# Autodesk Inventor assembly: TR1 Actuator
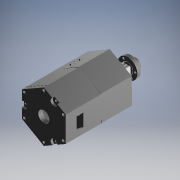
[picture p0: Inventor's stored thumbnail of the model, 180x180]
Saved by Autodesk Inventor 2017 (Build 210142000, 142)
## iProperties
Created: 2018-10-09
Part Number: TR1 Actuator
Document SubType Name: Assembly
Designer: Zach
Mass: 1249.01 g
Surface Area: 2931.11 cm^2
Volume: 1069.5 cm^3
Density: 1.16785 g/cm^3
Author: Zach
## Documents named in this file (21)
- C:\Users\Dell\Documents\GitHub\tr2\Actuator 1.3\Actuator 1.3.iam
- C:\Users\Dell\Documents\GitHub\tr2\Actuator 1.3\TA01.ipt
- C:\Users\Dell\Documents\GitHub\tr2\Actuator 1.3\Arm Actuator\Design Accelerator\Spur Gears2.iam
- C:\Users\Dell\Documents\GitHub\tr2\Actuator 1.3\EMS22XXX-D28-LSX.ipt
- C:\Users\Dell\Documents\GitHub\tr2\Actuator 1.3\12RPM Gear Motor.ipt
- C:\Users\Dell\Documents\GitHub\tr2\Actuator 1.3\Slip Ring.ipt
- C:\Users\Dell\Documents\GitHub\tr2\Actuator 1.3\TA06.ipt
- C:\Users\Dell\Documents\GitHub\tr2\Actuator 1.3\Steel Tubing.ipt
- C:\Users\Dell\Documents\GitHub\tr2\Actuator 1.3\Flange Bearing.ipt
- C:\Users\Dell\Documents\GitHub\tr2\Actuator 1.3\Shaft Collar.ipt
- C:\Users\Dell\Documents\GitHub\tr2\Actuator 1.3\Arm Actuator\Design Accelerator\Spur Gear13.ipt
- C:\Users\Dell\Documents\GitHub\tr2\Actuator 1.3\6mm Mounting Hub, thick.ipt
- C:\Users\Dell\Documents\GitHub\tr2\Actuator 1.3\TA02c.ipt
- C:\Users\Dell\Documents\GitHub\tr2\Actuator 1.3\TA02b.ipt
- C:\Users\Dell\Documents\GitHub\tr2\Actuator 1.3\Bushing.ipt
- C:\Users\Dell\Documents\GitHub\tr2\Actuator 1.3\545340 assembly.iam
- C:\Users\Dell\Documents\GitHub\tr2\Actuator 1.3\TA07.ipt
- C:\Users\Dell\Documents\GitHub\tr2\Actuator 1.3\TA08.ipt
- C:\Users\Dell\Documents\GitHub\tr2\Actuator 1.3\Rubber Square 1 in.ipt
- C:\Users\Dell\Documents\GitHub\tr2\Actuator 1.3\TA11.ipt
- C:\Users\Dell\Documents\Inventor\Content Center Files\R2017\en-US\ISO 4762(2)\ISO 4762 - M4 x 8ISO.ipt
## Components (26 placed, 20 different names)
1. TA01:1 — Mate:130, Mate:161, Mate:184, Mate:197, Mate:198, Mate:199
2. TA06:1 — Mate:34, Mate:35, Mate:82, Mate:83, Mate:129
3. Spur Gears:1 [sub-assembly] — Mate:33, Mate:97, Mate:121, Mate:123, Mate:124, Mate:125, Mate:129
4. 12RPM Gear Motor:1 — Mate:86, Mate:88, Mate:102, Mate:103, Mate:114, Mate:115
5. EMS22XXX-D28-LSX:1 — Mate:118, Mate:126, Angle:1, Mate:134, Mate:203
6. Slip Ring:1 — Mate:33, Mate:34, Mate:35, Mate:83
7. Steel Tubing:1 — Mate:76, Mate:77, Flush:2, Mate:82, Mate:84, Mate:96, Mate:98, Mate:104, Mate:120, Mate:121, Mate:162
8. Flange Bearing:1 — Mate:76, Mate:179
9. Shaft Collar:1 — Mate:77, Flush:2, Mate:180
10. Flange Bearing:2 — Mate:84, Mate:180
11. Spur Gear1:1 — Mate:88, Mate:116
12. 6mm Mounting Hub, thick:1 — Mate:86, Mate:114, Mate:116, Flush:3
13. TA02c:1 — Mate:98, Mate:99, Mate:105, Mate:127, Mate:128, Mate:130, Mate:131, Angle:2, Mate:197, Mate:198, Mate:199
14. TA02b:1 — Mate:96, Mate:97, Mate:99, Mate:102, Mate:103, Mate:115, Mate:126, Angle:1, Mate:131, Mate:132, Mate:133, Mate:134, Mate:179, Mate:185, Mate:187, Mate:188, Mate:189, Mate:190, Mate:191, Mate:193, Mate:194, Mate:195, Mate:196
15. Bushing:1 — Mate:104, Mate:105
16. Spur Gear1:2 — Mate:119
17. 6mm Mounting Hub, thick:2 — Mate:118, Mate:119, Flush:3, Mate:202
18. 545340 assembly:1 [sub-assembly] — Mate:120, Mate:123, Mate:124, Mate:125
19. EMS22XXX-D28-LSX:2 — Mate:127, Mate:128, Angle:2, Mate:135
20. TA07:1 — Mate:132, Mate:133, Mate:136, Mate:183
21. TA08:1 — Mate:135, Mate:136, Mate:183
22. Rubber Square 1 in:1 — Mate:192, Mate:193, Mate:194
23. Rubber Square 1 in:2 — Mate:186, Mate:195, Mate:196
24. TA11:1 — Mate:185, Mate:186, Mate:187, Mate:188
25. TA11:2 — Mate:189, Mate:190, Mate:191, Mate:192
26. ISO 4762 M4 x 8:2 — Mate:202, Mate:203
## Relationships (67: Mate 63, Flush 2, Angle 2)
- Mate:33: Spur Gears:1 ↔ Slip Ring:1
- Mate:34: TA06:1 ↔ Slip Ring:1
- Mate:35: TA06:1 ↔ Slip Ring:1
- Mate:76: Steel Tubing:1 ↔ Flange Bearing:1
- Mate:77: Steel Tubing:1 ↔ Shaft Collar:1
- Flush:2: Steel Tubing:1 ↔ Shaft Collar:1
- Mate:82: TA06:1 ↔ Steel Tubing:1
- Mate:83: TA06:1 ↔ Slip Ring:1
- Mate:84: Steel Tubing:1 ↔ Flange Bearing:2
- Mate:86: 12RPM Gear Motor:1 ↔ 6mm Mounting Hub, thick:1
- Mate:88: 12RPM Gear Motor:1 ↔ Spur Gear1:1
- Mate:96: Steel Tubing:1 ↔ TA02b:1
- Mate:97: Spur Gears:1 ↔ TA02b:1
- Mate:98: Steel Tubing:1 ↔ TA02c:1
- Mate:99: TA02c:1 ↔ TA02b:1
- Mate:102: 12RPM Gear Motor:1 ↔ TA02b:1
- Mate:103: 12RPM Gear Motor:1 ↔ TA02b:1
- Mate:104: Steel Tubing:1 ↔ Bushing:1
- Mate:105: TA02c:1 ↔ Bushing:1
- Mate:114: 12RPM Gear Motor:1 ↔ 6mm Mounting Hub, thick:1
- Mate:115: 12RPM Gear Motor:1 ↔ TA02b:1
- Mate:116: Spur Gear1:1 ↔ 6mm Mounting Hub, thick:1
- [Mate]: Spur Gear1:2 ↔ 6mm Mounting Hub, thick:2
- Mate:118: EMS22XXX-D28-LSX:1 ↔ 6mm Mounting Hub, thick:2
- Mate:119: Spur Gear1:2 ↔ 6mm Mounting Hub, thick:2
- Flush:3: 6mm Mounting Hub, thick:1 ↔ 6mm Mounting Hub, thick:2
- Mate:120: Steel Tubing:1 ↔ 545340 assembly:1
- Mate:121: Spur Gears:1 ↔ Steel Tubing:1
- Mate:123: Spur Gears:1 ↔ 545340 assembly:1
- Mate:124: Spur Gears:1 ↔ 545340 assembly:1
- Mate:125: Spur Gears:1 ↔ 545340 assembly:1
- Mate:126: EMS22XXX-D28-LSX:1 ↔ TA02b:1
- Angle:1 (0 deg): EMS22XXX-D28-LSX:1 ↔ TA02b:1
- Mate:127: TA02c:1 ↔ EMS22XXX-D28-LSX:2
- Mate:128: TA02c:1 ↔ EMS22XXX-D28-LSX:2
- Mate:129: TA06:1 ↔ Spur Gears:1
- Mate:130: TA01:1 ↔ TA02c:1
- Mate:131: TA02c:1 ↔ TA02b:1
- Angle:2 (0 deg): TA02c:1 ↔ EMS22XXX-D28-LSX:2
- Mate:132: TA02b:1 ↔ TA07:1
- Mate:133: TA02b:1 ↔ TA07:1
- Mate:134: EMS22XXX-D28-LSX:1 ↔ TA02b:1
- Mate:135: EMS22XXX-D28-LSX:2 ↔ TA08:1
- Mate:136: TA07:1 ↔ TA08:1
- Mate:161: TA01:1
- Mate:162: Steel Tubing:1
- Mate:179: Flange Bearing:1 ↔ TA02b:1
- Mate:180: Shaft Collar:1 ↔ Flange Bearing:2
- Mate:183: TA07:1 ↔ TA08:1
- Mate:184: TA01:1
- Mate:185: TA02b:1 ↔ TA11:1
- Mate:186: Rubber Square 1 in:2 ↔ TA11:1
- Mate:187: TA02b:1 ↔ TA11:1
- Mate:188: TA02b:1 ↔ TA11:1
- Mate:189: TA02b:1 ↔ TA11:2
- Mate:190: TA02b:1 ↔ TA11:2
- Mate:191: TA02b:1 ↔ TA11:2
- Mate:192: Rubber Square 1 in:1 ↔ TA11:2
- Mate:193: TA02b:1 ↔ Rubber Square 1 in:1
- Mate:194: TA02b:1 ↔ Rubber Square 1 in:1
- Mate:195: TA02b:1 ↔ Rubber Square 1 in:2
- Mate:196: TA02b:1 ↔ Rubber Square 1 in:2
- Mate:197: TA01:1 ↔ TA02c:1
- Mate:198: TA01:1 ↔ TA02c:1
- Mate:199: TA01:1 ↔ TA02c:1
- Mate:202: 6mm Mounting Hub, thick:2 ↔ ISO 4762 M4 x 8:2
- Mate:203 (-16 mm): EMS22XXX-D28-LSX:1 ↔ ISO 4762 M4 x 8:2
## Named parameters: d140_d139 = 0 mm
